# Autodesk Inventor assembly: Mitutoyo-5pos-726
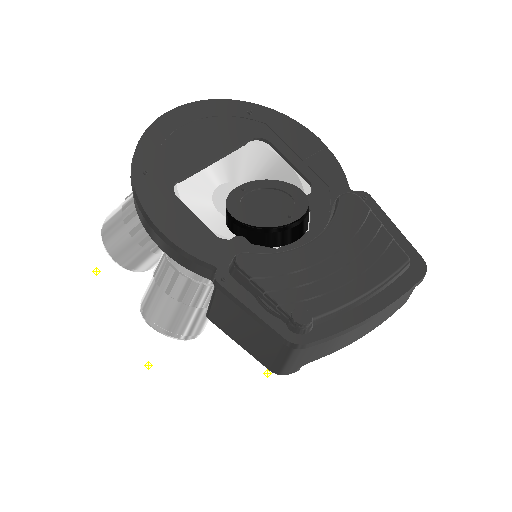
[picture p0: Inventor's stored thumbnail of the model, 512x512]
Saved by Autodesk Inventor 2023 (Build 270158000, 158)
## iProperties
Created: 2023-01-18
Part Number: Mitutoyo-5pos-726
Document SubType Name: Assembly
Designer: nvladi
Author: nvladi
## Documents named in this file (3)
- C:\Users\Public\GitHub-public\benchtop-hardware\v4-5-upgrade-2023\CAD-AutodeskInventor2021\Mitutoyo-5pos-726.iam
- C:\Users\Public\GitHub-public\benchtop-hardware\Benchtop\CAD-model-Inventor\library\Mitutoyo\BD-Plan-Apo-approx.ipt
- C:\Users\Public\CAD\Mitutoyo-turrets\WIDE_BF-P-REVO_378-726.iam
## Components (6 placed, 2 different names)
1. WIDE_BF-P-REVO_378-726:1 [sub-assembly] — Insert:1, Insert:2, Insert:3, Insert:4, Insert:5
2. BD-Plan-Apo-approx:1 — Insert:1
3. BD-Plan-Apo-approx:2 — Insert:4
4. BD-Plan-Apo-approx:3 — Insert:3
5. BD-Plan-Apo-approx:4 — Insert:5
6. BD-Plan-Apo-approx:5 — Insert:2
## Relationships (5: Insert 5)
- Insert:1: WIDE_BF-P-REVO_378-726:1 ↔ BD-Plan-Apo-approx:1
- Insert:2: WIDE_BF-P-REVO_378-726:1 ↔ BD-Plan-Apo-approx:5
- Insert:3: WIDE_BF-P-REVO_378-726:1 ↔ BD-Plan-Apo-approx:3
- Insert:4: WIDE_BF-P-REVO_378-726:1 ↔ BD-Plan-Apo-approx:2
- Insert:5: WIDE_BF-P-REVO_378-726:1 ↔ BD-Plan-Apo-approx:4
